# Autodesk Inventor assembly: SC-0-01-Science apparatus
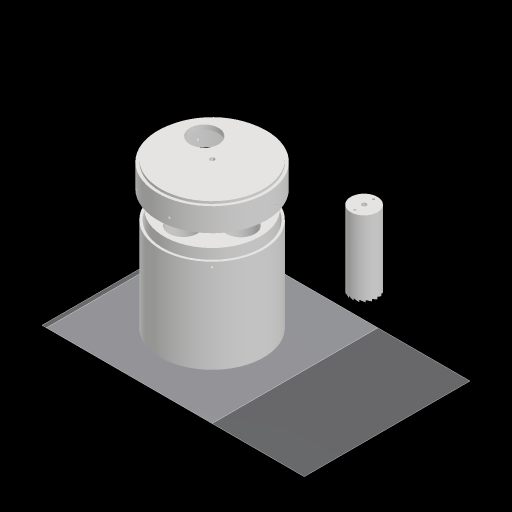
[picture p0: Inventor's stored thumbnail of the model, 512x512]
Saved by Autodesk Inventor 2023 (Build 270158000, 158)
## iProperties
Created: 2024-01-01
Part Number: SC-0-01-Science apparatus
Document SubType Name: Assembly
Designer: annah
Author: annah
## Documents named in this file (3)
- C:\Users\annah\Documents\GitHub\BehrendURCMechanical\CAD\Science\SC-0-01-Science apparatus.iam
- C:\Users\annah\Documents\GitHub\BehrendURCMechanical\CAD\Science\SC-0-01-ICE Assembly.iam
- C:\Users\annah\Documents\GitHub\BehrendURCMechanical\CAD\Science\SC-1-01- Hole Saw.ipt
## Components (2 placed, 2 different names)
1. SC-0-01-ICE Assembly:1 [sub-assembly] — Mate:1
2. SC-1-01- Hole Saw:1
## Relationships (1: Mate 1)
- Mate:1: SC-0-01-ICE Assembly:1
